# Autodesk Inventor assembly: DriveTrainFrame
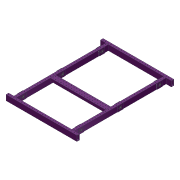
[picture p0: Inventor's stored thumbnail of the model, 180x180]
Saved by Autodesk Inventor 2012 (Build 160160000, 160)
## iProperties
Created: 2012-11-17
Part Number: DriveTrainFrame
Document SubType Name: Assembly
Designer: JesseK
Mass: 4313.77 g
Surface Area: 9857.05 cm^2
Volume: 1591.8 cm^3
Density: 2.71 g/cm^3
Author: JesseK
## Documents named in this file (5)
- Z:\UserData\Documents\Inventor\team1885frc\Robot2013\DriveTrainProto\DriveTrainFrame.iam
- Z:\UserData\Documents\Inventor\team1885frc\Robot2013\DriveTrainProto\SideRail.ipt
- Z:\UserData\Documents\Inventor\team1885frc\Robot2013\DriveTrainProto\BearingBlockAssembly.iam
- Z:\UserData\Documents\Inventor\team1885frc\Robot2013\DriveTrainProto\OuterCrossRail.ipt
- Z:\UserData\Documents\Inventor\team1885frc\Robot2013\DriveTrainProto\InnerCrossRail.ipt
## Components (11 placed, 4 different names)
1. SideRail:1 — Mate:1, Mate:2, Mate:3, Mate:4, Mate:5, Mate:6, Mate:13, Mate:16, Flush:1, Mate:19, Mate:20, Mate:29
2. SideRail:2 — Mate:7, Mate:8, Mate:9, Mate:10, Mate:11, Mate:12, Mate:14, Mate:15, Mate:21, Flush:2, Flush:3, Mate:22, Mate:23, Mate:25, Mate:28
3. BearingBlockAssembly:1 [sub-assembly] — Mate:9, Mate:10, Mate:14
4. BearingBlockAssembly:2 [sub-assembly] — Mate:7, Mate:12, Mate:15
5. BearingBlockAssembly:3 [sub-assembly] — Mate:2, Mate:5, Mate:27
6. BearingBlockAssembly:4 [sub-assembly] — Mate:3, Mate:4, Mate:16
7. BearingBlockAssembly:5 [sub-assembly] — Mate:8, Mate:11, Mate:27, Mate:28
8. BearingBlockAssembly:6 [sub-assembly] — Mate:1, Mate:6, Mate:13
9. OuterCrossRail:1 — Mate:22, Mate:23, Mate:24
10. OuterCrossRail:2 — Flush:1, Mate:19, Mate:20, Mate:21, Flush:2, Flush:3, Mate:24
11. InnerCrossRail:1 — Mate:25, Mate:29
## Relationships (29: Mate 26, Flush 3)
- Mate:1: SideRail:1 ↔ BearingBlockAssembly:6
- Mate:2: SideRail:1 ↔ BearingBlockAssembly:3
- Mate:3: SideRail:1 ↔ BearingBlockAssembly:4
- Mate:4: SideRail:1 ↔ BearingBlockAssembly:4
- Mate:5: SideRail:1 ↔ BearingBlockAssembly:3
- Mate:6: SideRail:1 ↔ BearingBlockAssembly:6
- Mate:7: SideRail:2 ↔ BearingBlockAssembly:2
- Mate:8: SideRail:2 ↔ BearingBlockAssembly:5
- Mate:9: SideRail:2 ↔ BearingBlockAssembly:1
- Mate:10: SideRail:2 ↔ BearingBlockAssembly:1
- Mate:11: SideRail:2 ↔ BearingBlockAssembly:5
- Mate:12: SideRail:2 ↔ BearingBlockAssembly:2
- Mate:13: SideRail:1 ↔ BearingBlockAssembly:6
- Mate:14: SideRail:2 ↔ BearingBlockAssembly:1
- Mate:15: SideRail:2 ↔ BearingBlockAssembly:2
- Mate:16: SideRail:1 ↔ BearingBlockAssembly:4
- Flush:1 (-50.8 mm): SideRail:1 ↔ OuterCrossRail:2
- Mate:19: SideRail:1 ↔ OuterCrossRail:2
- Mate:20: SideRail:1 ↔ OuterCrossRail:2
- Mate:21: SideRail:2 ↔ OuterCrossRail:2
- Flush:2: SideRail:2 ↔ OuterCrossRail:2
- Flush:3 (50.8 mm): SideRail:2 ↔ OuterCrossRail:2
- Mate:22: SideRail:2 ↔ OuterCrossRail:1
- Mate:23: SideRail:2 ↔ OuterCrossRail:1
- Mate:24: OuterCrossRail:1 ↔ OuterCrossRail:2
- Mate:25: SideRail:2 ↔ InnerCrossRail:1
- Mate:27: BearingBlockAssembly:3 ↔ BearingBlockAssembly:5
- Mate:28: SideRail:2 ↔ BearingBlockAssembly:5
- Mate:29: SideRail:1 ↔ InnerCrossRail:1
